# Autodesk Inventor assembly: 176-DP(F,D-231-1)
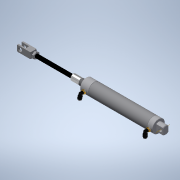
[picture p0: Inventor's stored thumbnail of the model, 180x180]
Saved by Autodesk Inventor 2020 (Build 240168000, 168)
## iProperties
Created: 2020-02-18
Part Number: 176-DP(F,D-231-1)
Catalog Web Link: www.cadenas.de
Description: Original Line Standard Air Cylinders-Standard Air Cylinders
Vendor: BIMBA
Document SubType Name: Assembly
Designer: psadmin
Manufacturer: BIMBA
Mass: 680.389 g
Surface Area: 873.052 cm^2
Volume: 138.889 cm^3
Density: 4.89881 g/cm^3
Category: PARTsolutions
Company: BIMBA
Title: 176-DP
Author: Cadenas PARTsolutions
Comments: Standard Air Cylinders
## Documents named in this file (11)
- T:\EIT\2022 Rapid React\COMMON PARTS\AIR CYLINDERS\176-DP\AIS2018\176-DP(F,D-231-1).iam
- T:\EIT\2022 Rapid React\COMMON PARTS\AIR CYLINDERS\176-DP\AIS2018\176-DPC(F,D-231-1)0000000_0_dummy.ipt
- T:\EIT\2022 Rapid React\COMMON PARTS\AIR CYLINDERS\176-DP\AIS2018\17R000-0_rod_guide.ipt
- T:\EIT\2022 Rapid React\COMMON PARTS\AIR CYLINDERS\176-DP\AIS2018\17R-7_30250C.ipt
- T:\EIT\2022 Rapid React\COMMON PARTS\AIR CYLINDERS\176-DP\AIS2018\17P0000_rear_head.ipt
- T:\EIT\2022 Rapid React\COMMON PARTS\AIR CYLINDERS\176-DP\AIS2018\C-176-DP0000_rod.ipt
- T:\EIT\2022 Rapid React\COMMON PARTS\AIR CYLINDERS\176-DP\AIS2018\D-231-1-dummy.ipt
- T:\EIT\2022 Rapid React\COMMON PARTS\AIR CYLINDERS\176-DP\AIS2018\D-14053.ipt
- T:\EIT\2022 Rapid React\COMMON PARTS\AIR CYLINDERS\5779K151_PUSH-TO-CONNECT TUBE FITTING FOR AIR.ipt
- T:\EIT\2022 Rapid React\COMMON PARTS\AIR CYLINDERS\176-DP\AIS2018\D-154.ipt
- T:\EIT\2022 Rapid React\CLIMBER\Spacers\CL-S-011.ipt
## Components (11 placed, 10 different names)
1. 176-DPC(F,D-231-1)0000000_0_dummy:1
2. 17R000-0_rod_guide:1 — Insert:1, Insert:8, Insert:11
3. 17R-7_30250C:1
4. 17P0000_rear_head:1 — Angle:1, Mate:1, Insert:7
5. C-176-DP0000_rod:1 — Insert:1, Insert:9
6. D-231-1-dummy:1
7. D-14053:1 — Angle:1, Insert:10
8. 5779K151_PUSH-TO-CONNECT TUBE FITTING FOR AIR:1 — Insert:7
9. 5779K151_PUSH-TO-CONNECT TUBE FITTING FOR AIR:2 — Insert:8
10. D-154:1 — Insert:9, Insert:10
11. CL-S-011:1 — Insert:11
## Relationships (8: Insert 6, Angle 1, Mate 1)
- Insert:1: 17R000-0_rod_guide:1 ↔ C-176-DP0000_rod:1
- Angle:1 (0 deg): 17P0000_rear_head:1 ↔ D-14053:1
- Mate:1: 17P0000_rear_head:1
- Insert:7 (9.525 mm): 17P0000_rear_head:1 ↔ 5779K151_PUSH-TO-CONNECT TUBE FITTING FOR AIR:1
- Insert:8 (6.35 mm): 17R000-0_rod_guide:1 ↔ 5779K151_PUSH-TO-CONNECT TUBE FITTING FOR AIR:2
- Insert:9: C-176-DP0000_rod:1 ↔ D-154:1
- Insert:10 (3.175 mm): D-14053:1 ↔ D-154:1
- Insert:11: 17R000-0_rod_guide:1 ↔ CL-S-011:1
